# Autodesk Inventor assembly: Drakon 1.75mm
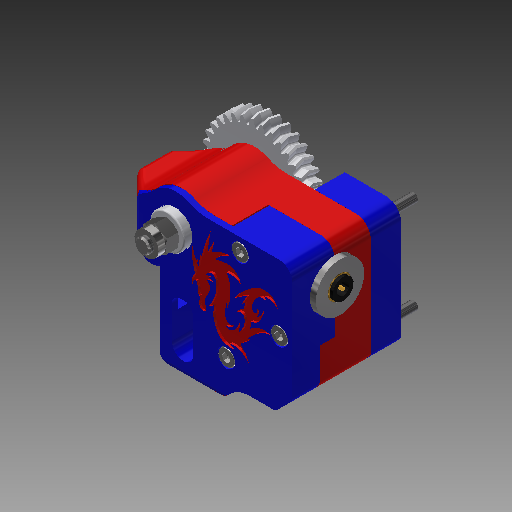
[picture p0: Inventor's stored thumbnail of the model, 512x512]
Saved by Autodesk Inventor 2019 (Build 230136000, 136)
## iProperties
Created: 2018-09-06
Part Number: Drakon 1.75mm
Document SubType Name: Assembly
Designer: Ax
Author: Ax
## Documents named in this file (19)
- C:\Users\Ax\Google Drive\Inventor\Library\Drakon\Drakon 1.75mm.iam
- C:\Users\Ax\Google Drive\Inventor\Library\Drakon\RAMPSDrakon_1.75_Body.ipt
- C:\Users\Ax\Google Drive\Inventor\Library\Drakon\RAMPSDrakon_1.75_Cover.ipt
- C:\Users\Ax\Google Drive\Inventor\Library\Drakon\RAMPSDrakon_1.75_Idler.ipt
- C:\Users\Ax\Google Drive\Inventor\Library\Drakon\RAMPSDrakon_Base.ipt
- C:\Users\Ax\Google Drive\Inventor\Library\Drakon\RAMPSDrakon_Small_Gear.ipt
- C:\Users\Ax\Google Drive\Inventor\Library\Drakon\RAMPSDrakon_Large_Gear.ipt
- C:\Users\Ax\Google Drive\Inventor\Library\625ZZ.ipt
- C:\Users\Ax\Google Drive\Inventor\Library\MK8.ipt
- C:\Users\Ax\Google Drive\Inventor\Library\Drakon\Drakon_Spindle_Bushing.ipt
- C:\Users\Ax\Google Drive\Inventor\Library\Drakon\Drakon_1.75_Filament_Guide.ipt
- C:\Users\Ax\Google Drive\Inventor\Library\Drakon\Compress Spring1.iam
- C:\Users\Ax\Google Drive\Autodesk\Content Center Files\R2017\en-US\DIN 931-1\DIN 931-1 - M5 x 40.ipt
- C:\Users\Ax\Google Drive\Autodesk\Content Center Files\R2017\en-US\SS-ISO 7040\SS-ISO 7040 - M5.ipt
- C:\Users\Ax\Google Drive\Autodesk\Content Center Files\R2017\en-US\DIN 912\DIN 912 - M3 x 0.5 x 30 x 18.ipt
- C:\Users\Ax\Google Drive\Autodesk\Content Center Files\R2017\en-US\DIN 934\DIN 934 - M3 x 0.5.ipt
- C:\Users\Ax\Google Drive\Autodesk\Content Center Files\R2017\en-US\DIN 912\DIN 912 - M4 x 0.7 x 20 x 18.25.ipt
- C:\Users\Ax\Google Drive\Autodesk\Content Center Files\R2017\en-US\DIN 912\DIN 912 - M3 x 0.5 x 16 x 14.75.ipt
- C:\Users\Ax\Google Drive\Inventor\Library\Drakon\Groove_Mount_Adaptor_1_75.iam
## Components (27 placed, 18 different names)
1. Drakon_1.75_Body:1 — Rigid:1, Rotational:4, Mate:10, Mate:11, Mate:12, Mate:13, Mate:14, Rotational:6, Mate:15, Mate:16, Mate:17, Mate:18, Mate:19, Insert:4, Insert:7, Mate:28, Mate:29, Mate:30, Mate:33, Mate:35
2. RAMPSDrakon_1.75_Cover:1 — Rigid:1, Mate:10, Mate:11, Mate:12, Cylindrical:1, Insert:1, Insert:2, Insert:3, Mate:31
3. RAMPSDrakon_1.75_Idler:1 — Rotational:4
4. RAMPSDrakon_Base:1 — Insert:5, Insert:6, Insert:9, Insert:10, Insert:11, Mate:28, Mate:29, Mate:30, Mate:34, Flush:1
5. RAMPSDrakon_Small_Gear:1 — Rotational:6
6. RAMPSDrakon_Large_Gear:1 — Rotational:7, Mate:21, Mate:22, Mate:23
7. 625ZZ:1 — Mate:14, Rotational:7, Mate:15, Rotational:8
8. 625ZZ:2 — Mate:13, Mate:16
9. MK8:1 — Rotational:8, Rotational:9
10. Drakon_Spindle_Bushing:1 — Rotational:9
11. Drakon_Spindle_Bushing:2 — Cylindrical:1, Mate:25, Mate:31
12. Drakon_1.75_Filament_Guide:1 — Mate:17, Mate:18, Mate:19, Mate:26, Mate:27
13. Compress Spring:1 [sub-assembly] — Mate:32, Mate:33
14. DIN 931-1 - replaced by DIN EN 24014 M5 x 40:1 — Mate:21, Mate:22, Mate:23, Mate:24
15. SS ISO 7040 M5:1 — Mate:24, Mate:25
16. DIN 912 - replaced by DIN EN ISO 4762 M3 x 30:1 — Insert:3
17. DIN 912 - replaced by DIN EN ISO 4762 M3 x 30:2 — Insert:2
18. DIN 912 - replaced by DIN EN ISO 4762 M3 x 30:3 — Insert:1
19. DIN 934 - replaced by DIN EN 24032/28673/28674 M3:1 — Insert:6
20. DIN 934 - replaced by DIN EN 24032/28673/28674 M3:2 — Insert:5
21. DIN 934 - replaced by DIN EN 24032/28673/28674 M3:3 — Insert:4
22. DIN 912 - replaced by DIN EN ISO 4762 M4 x 20:1 — Insert:7, Insert:8, Mate:32
23. DIN 934 - replaced by DIN EN 24032/28673/28674 M3:4 — Insert:8
24. DIN 912 - replaced by DIN EN ISO 4762 M3 x 16:1 — Insert:9
25. DIN 912 - replaced by DIN EN ISO 4762 M3 x 16:2 — Insert:10
26. DIN 912 - replaced by DIN EN ISO 4762 M3 x 16:3 — Insert:11
27. Groove_Mount_Adaptor_1_75:1 [sub-assembly] — Mate:26, Mate:27
## Relationships (44: Mate 25, Insert 11, RevoluteJoint 5, WeldJoint 1, CylindricalJoint 1, Flush 1)
- Rigid:1 [WeldJoint]: Drakon_1.75_Body:1 ↔ RAMPSDrakon_1.75_Cover:1
- Rotational:4 [RevoluteJoint]: Drakon_1.75_Body:1 ↔ RAMPSDrakon_1.75_Idler:1
- Mate:10: Drakon_1.75_Body:1 ↔ RAMPSDrakon_1.75_Cover:1
- Mate:11: Drakon_1.75_Body:1 ↔ RAMPSDrakon_1.75_Cover:1
- Mate:12: Drakon_1.75_Body:1 ↔ RAMPSDrakon_1.75_Cover:1
- Mate:13: Drakon_1.75_Body:1 ↔ 625ZZ:2
- Mate:14: Drakon_1.75_Body:1 ↔ 625ZZ:1
- Rotational:6 [RevoluteJoint] (-1.25 mm): Drakon_1.75_Body:1 ↔ RAMPSDrakon_Small_Gear:1
- Rotational:7 [RevoluteJoint] (-1.5 mm): RAMPSDrakon_Large_Gear:1 ↔ 625ZZ:1
- Mate:15: Drakon_1.75_Body:1 ↔ 625ZZ:1
- Mate:16: Drakon_1.75_Body:1 ↔ 625ZZ:2
- Rotational:8 [RevoluteJoint] (-0.75 mm): 625ZZ:1 ↔ MK8:1
- Rotational:9 [RevoluteJoint]: MK8:1 ↔ Drakon_Spindle_Bushing:1
- Cylindrical:1: RAMPSDrakon_1.75_Cover:1 ↔ Drakon_Spindle_Bushing:2
- Mate:17: Drakon_1.75_Body:1 ↔ Drakon_1.75_Filament_Guide:1
- Mate:18: Drakon_1.75_Body:1 ↔ Drakon_1.75_Filament_Guide:1
- Mate:19: Drakon_1.75_Body:1 ↔ Drakon_1.75_Filament_Guide:1
- Mate:21: RAMPSDrakon_Large_Gear:1 ↔ DIN 931-1 - replaced by DIN EN 24014 M5 x 40:1
- Mate:22: RAMPSDrakon_Large_Gear:1 ↔ DIN 931-1 - replaced by DIN EN 24014 M5 x 40:1
- Mate:23: RAMPSDrakon_Large_Gear:1 ↔ DIN 931-1 - replaced by DIN EN 24014 M5 x 40:1
- Mate:24: DIN 931-1 - replaced by DIN EN 24014 M5 x 40:1 ↔ SS ISO 7040 M5:1
- Mate:25: Drakon_Spindle_Bushing:2 ↔ SS ISO 7040 M5:1
- Insert:1: RAMPSDrakon_1.75_Cover:1 ↔ DIN 912 - replaced by DIN EN ISO 4762 M3 x 30:3
- Insert:2: RAMPSDrakon_1.75_Cover:1 ↔ DIN 912 - replaced by DIN EN ISO 4762 M3 x 30:2
- Insert:3: RAMPSDrakon_1.75_Cover:1 ↔ DIN 912 - replaced by DIN EN ISO 4762 M3 x 30:1
- Insert:4: Drakon_1.75_Body:1 ↔ DIN 934 - replaced by DIN EN 24032/28673/28674 M3:3
- Insert:5: RAMPSDrakon_Base:1 ↔ DIN 934 - replaced by DIN EN 24032/28673/28674 M3:2
- Insert:6: RAMPSDrakon_Base:1 ↔ DIN 934 - replaced by DIN EN 24032/28673/28674 M3:1
- Insert:7: Drakon_1.75_Body:1 ↔ DIN 912 - replaced by DIN EN ISO 4762 M4 x 20:1
- Insert:8 (-4.4 mm): DIN 912 - replaced by DIN EN ISO 4762 M4 x 20:1 ↔ DIN 934 - replaced by DIN EN 24032/28673/28674 M3:4
- Insert:9: RAMPSDrakon_Base:1 ↔ DIN 912 - replaced by DIN EN ISO 4762 M3 x 16:1
- Insert:10: RAMPSDrakon_Base:1 ↔ DIN 912 - replaced by DIN EN ISO 4762 M3 x 16:2
- Insert:11: RAMPSDrakon_Base:1 ↔ DIN 912 - replaced by DIN EN ISO 4762 M3 x 16:3
- Mate:26: Drakon_1.75_Filament_Guide:1 ↔ Groove_Mount_Adaptor_1_75:1
- Mate:27: Drakon_1.75_Filament_Guide:1 ↔ Groove_Mount_Adaptor_1_75:1
- Mate:28: Drakon_1.75_Body:1 ↔ RAMPSDrakon_Base:1
- Mate:29: Drakon_1.75_Body:1 ↔ RAMPSDrakon_Base:1
- Mate:30: Drakon_1.75_Body:1 ↔ RAMPSDrakon_Base:1
- Mate:31: RAMPSDrakon_1.75_Cover:1 ↔ Drakon_Spindle_Bushing:2
- Mate:32: Compress Spring:1 ↔ DIN 912 - replaced by DIN EN ISO 4762 M4 x 20:1
- Mate:33 (1.7 mm): Drakon_1.75_Body:1 ↔ Compress Spring:1
- Mate:34: RAMPSDrakon_Base:1
- Mate:35: Drakon_1.75_Body:1
- Flush:1: RAMPSDrakon_Base:1
